# Autodesk Inventor assembly: ASY TZS FDS way3_940
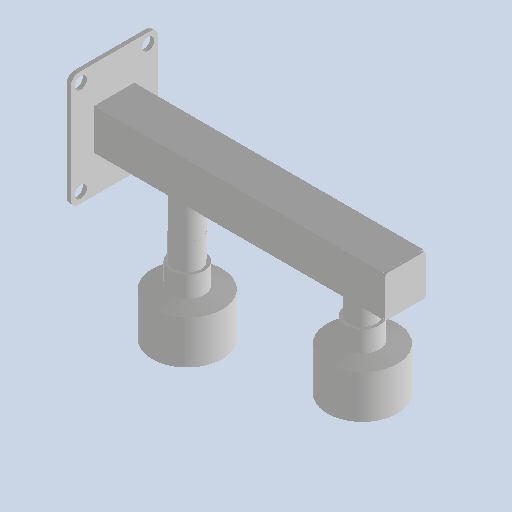
[picture p0: Inventor's stored thumbnail of the model, 512x512]
Saved by Autodesk Inventor 2025 (Build 290162010, 162A)
## iProperties
Created: 2025-07-02
Part Number: ASY TZS FDS way3_940
Document SubType Name: Assembly
Designer: admin
Author: user
## Documents named in this file (7)
- C:\Users\pokla\Documents\Inventor\TZS-Tazovskiy\Filter D940\FDS 940\ASY TZS FDS way3_940.iam
- C:\Users\pokla\Documents\Inventor\TZS-Tazovskiy\Filter D940\FDS 940\TZS 1663 FDS 940 way tube 3.ipt
- C:\Users\pokla\Documents\Inventor\TZS-Tazovskiy\Filter D940\FDS 940\TZS dummy filter element_940.ipt
- C:\Users\pokla\Documents\Inventor\TZS-Tazovskiy\Filter D940\FDS 940\TZS dummy pipe nippel_940.ipt
- C:\Users\pokla\Documents\Inventor\TZS-Tazovskiy\Filter D940\FDS 940\TZS 1687 FDS 940 way tube 7.ipt
- C:\Users\pokla\Documents\Inventor\TZS-Tazovskiy\Filter D940\FDS 940\TZS 1669 FDS 940 FLANGE 3.ipt
- C:\Users\pokla\Documents\Inventor\TZS-Tazovskiy\Filter D940\FDS 940\TZS 1666 FDS 940 CUP 1.ipt
## Components (8 placed, 6 different names)
1. TZS 1663 FDS 940 way tube 3.ipt:1 — Rigid:2, Rigid:5, Rigid:6, Rigid:7
2. TZS dummy filter element_940.ipt:1 — Rigid:1
3. TZS dummy pipe nippel_940.ipt:1 — Rigid:2, Rigid:1
4. TZS 1687 FDS 940 way tube 7.ipt:1 — Rigid:5, Rigid:4
5. TZS dummy filter element_940.ipt:2 — Rigid:3
6. TZS dummy pipe nippel_940.ipt:2 — Rigid:4, Rigid:3
7. TZS 1669 FDS 940 FLANGE 3.ipt:1 — Rigid:6
8. TZS 1666 FDS 940 CUP 1.ipt:1 — Rigid:7
## Relationships (7: WeldJoint 7)
- Rigid:2 [WeldJoint]: TZS 1663 FDS 940 way tube 3.ipt:1 ↔ TZS dummy pipe nippel_940.ipt:1
- Rigid:1 [WeldJoint]: TZS dummy filter element_940.ipt:1 ↔ TZS dummy pipe nippel_940.ipt:1
- Rigid:5 [WeldJoint]: TZS 1663 FDS 940 way tube 3.ipt:1 ↔ TZS 1687 FDS 940 way tube 7.ipt:1
- Rigid:4 [WeldJoint]: TZS 1687 FDS 940 way tube 7.ipt:1 ↔ TZS dummy pipe nippel_940.ipt:2
- Rigid:3 [WeldJoint]: TZS dummy filter element_940.ipt:2 ↔ TZS dummy pipe nippel_940.ipt:2
- Rigid:6 [WeldJoint] (-3 mm): TZS 1663 FDS 940 way tube 3.ipt:1 ↔ TZS 1669 FDS 940 FLANGE 3.ipt:1
- Rigid:7 [WeldJoint]: TZS 1663 FDS 940 way tube 3.ipt:1 ↔ TZS 1666 FDS 940 CUP 1.ipt:1
